# Autodesk Inventor assembly: Idler Assembly
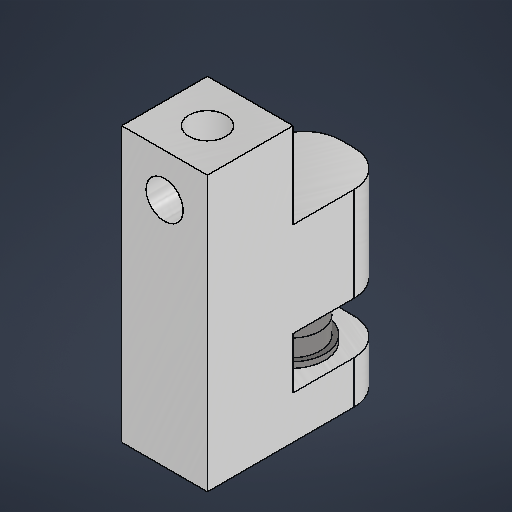
[picture p0: Inventor's stored thumbnail of the model, 512x512]
Saved by Autodesk Inventor 2026 (Build 300175050, 175E)
## iProperties
Created: 2025-05-27
Part Number: Idler Assembly
Document SubType Name: Assembly
Designer: Joshua Eah
Author: Joshua Eah
## Documents named in this file (5)
- C:\Users\Joshua Eah\Documents\GitHub\Voron-0\CAD\Tulip - Machined Parts\Idlers\Design 1\Idler Assembly.iam
- C:\Users\Joshua Eah\Documents\GitHub\Voron-0\CAD\Tulip - Machined Parts\Idlers\Design 1\A Idler (Tulip).ipt
- C:\Users\Joshua Eah\Documents\GitHub\Voron-0\CAD\Master Assembly\Hardware\F623 Stack.iam
- C:\Users\Joshua Eah\Documents\GitHub\Voron-0\CAD\Tulip - Machined Parts\Idlers\Design 1\Bearing Nut.ipt
- C:\Users\Joshua Eah\Documents\GitHub\Voron-0\CAD\Master Assembly\Hardware\3x12 Pin.ipt
## Components (5 placed, 4 different names)
1. A Idler (Tulip):1
2. Bearing Nut:1 — Mate:6, Insert:2
3. Bearing Nut:2 — Mate:5, Insert:1
4. 3x12 Pin:1 — Mate:5, Mate:6, Insert:1
5. F623 Stack:1 [sub-assembly] — Insert:2
## Relationships (4: Mate 2, Insert 2)
- Mate:5: Bearing Nut:2 ↔ 3x12 Pin:1
- Mate:6: Bearing Nut:1 ↔ 3x12 Pin:1
- Insert:1: Bearing Nut:2 ↔ 3x12 Pin:1
- Insert:2: Bearing Nut:1 ↔ F623 Stack:1
